# Autodesk Inventor assembly: Final assembly 3
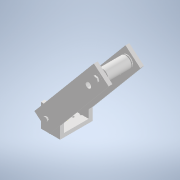
[picture p0: Inventor's stored thumbnail of the model, 180x180]
Saved by Autodesk Inventor 2022 (Build 260153000, 153)
## iProperties
Created: 2022-06-16
Part Number: Final assembly 3
Document SubType Name: Assembly
Designer: chait
Author: chait
## Documents named in this file (3)
- C:\Users\chait\Documents\Final assembly 3.iam
- C:\Users\chait\Documents\Final assembly 2.iam
- C:\Users\chait\Documents\Screw 3mm.ipt
## Components (3 placed, 2 different names)
1. Final assembly 2:1 [sub-assembly] — Insert:1, Insert:2
2. Screw 3mm:1 — Insert:1
3. Screw 3mm:2 — Insert:2
## Relationships (2: Insert 2)
- Insert:1: Final assembly 2:1 ↔ Screw 3mm:1
- Insert:2 (-13.9 mm): Final assembly 2:1 ↔ Screw 3mm:2
